# Autodesk Inventor assembly: Foot
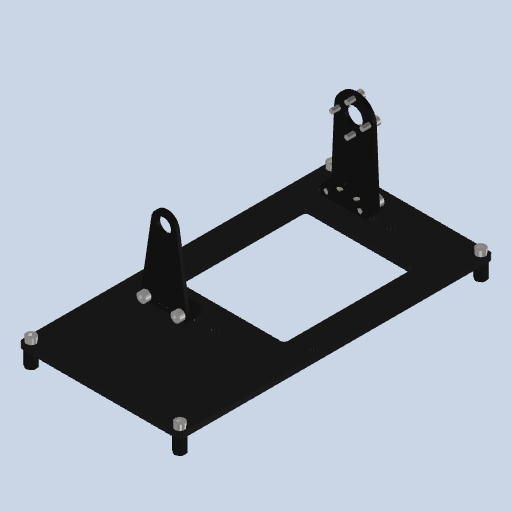
[picture p0: Inventor's stored thumbnail of the model, 512x512]
Saved by Autodesk Inventor 2022 (Build 260153000, 153)
## iProperties
Created: 2022-06-04
Part Number: Foot
Document SubType Name: Assembly
Designer: Masato Kubotera
Author: Masato Kubotera
## Documents named in this file (9)
- C:\Users\MasatoKubotera\Desktop\SUSTAINA-OP\LowerBody\Foot\Foot.iam
- C:\Users\MasatoKubotera\Desktop\SUSTAINA-OP\LowerBody\Foot\Foot_back_frame.ipt
- C:\Users\MasatoKubotera\Desktop\SUSTAINA-OP\LowerBody\Foot\Foot_front_frame.ipt
- C:\Users\MasatoKubotera\Desktop\SUSTAINA-OP\LowerBody\Foot\Foot_root_block.ipt
- C:\Users\MasatoKubotera\Desktop\SUSTAINA-OP\LowerBody\Foot\Sole_frame.ipt
- C:\Users\MasatoKubotera\Desktop\SUSTAINA-OP\ReadyMade\Screw\UC-0308.ipt
- C:\Users\MasatoKubotera\Desktop\SUSTAINA-OP\ReadyMade\Screw\UC-2606.ipt
- C:\Users\MasatoKubotera\Desktop\SUSTAINA-OP\ReadyMade\Spacer\ASL-309BE.ipt
- C:\Users\MasatoKubotera\Desktop\SUSTAINA-OP\ReadyMade\Screw\UC-0310.ipt
## Components (25 placed, 8 different names)
1. Sole_frame:1 — 挿入:1, 挿入:2, 挿入:3, 挿入:4, 挿入:13, 挿入:14, 挿入:15, 挿入:16, 挿入:21, 挿入:22, 挿入:23, 挿入:24, 挿入:25, 挿入:26, 挿入:27, 挿入:28
2. Foot_front_frame:1 — 挿入:5, 挿入:6, メイト:1, メイト:2, 挿入:31, 挿入:32
3. Foot_back_frame:1 — 挿入:7, 挿入:8, 挿入:17, 挿入:18, 挿入:19, 挿入:20, 挿入:29, 挿入:30
4. Foot_root_block:1 — 挿入:1, 挿入:2, 挿入:5, 挿入:6
5. Foot_root_block:2 — 挿入:3, 挿入:4, 挿入:7, 挿入:8
6. ASL-309BE:1 — 挿入:21, メイト:3, 角度:1
7. ASL-309BE:2 — 挿入:22, 角度:2
8. ASL-309BE:3 — 挿入:23, 角度:3
9. ASL-309BE:4 — 挿入:24, 角度:4
10. UC-0308:5 — 挿入:32
11. UC-0308:6 — 挿入:31
12. UC-0308:7 — 挿入:29
13. UC-0308:8 — 挿入:30
14. UC-0310:1 — 挿入:25
15. UC-0310:2 — 挿入:26
16. UC-0310:3 — 挿入:27
17. UC-0310:4 — 挿入:28
18. UC-0308:1 — 挿入:13
19. UC-0308:2 — 挿入:14
20. UC-0308:3 — 挿入:15
21. UC-0308:4 — 挿入:16
22. UC-2606:1 — 挿入:17
23. UC-2606:2 — 挿入:18
24. UC-2606:3 — 挿入:19
25. UC-2606:4 — 挿入:20
## Relationships (35: Insert 28, Angle 4, Mate 3)
- メイト:1 [Mate]: Foot_front_frame:1
- メイト:2 [Mate]: Foot_front_frame:1
- メイト:3 [Mate]: ASL-309BE:1
- 挿入:1 [Insert]: Sole_frame:1 ↔ Foot_root_block:1
- 挿入:2 [Insert]: Sole_frame:1 ↔ Foot_root_block:1
- 挿入:3 [Insert]: Sole_frame:1 ↔ Foot_root_block:2
- 挿入:4 [Insert]: Sole_frame:1 ↔ Foot_root_block:2
- 挿入:5 [Insert]: Foot_front_frame:1 ↔ Foot_root_block:1
- 挿入:6 [Insert]: Foot_front_frame:1 ↔ Foot_root_block:1
- 挿入:7 [Insert]: Foot_back_frame:1 ↔ Foot_root_block:2
- 挿入:8 [Insert]: Foot_back_frame:1 ↔ Foot_root_block:2
- 挿入:13 [Insert]: Sole_frame:1 ↔ UC-0308:1
- 挿入:14 [Insert]: Sole_frame:1 ↔ UC-0308:2
- 挿入:15 [Insert]: Sole_frame:1 ↔ UC-0308:3
- 挿入:16 [Insert]: Sole_frame:1 ↔ UC-0308:4
- 挿入:17 [Insert]: Foot_back_frame:1 ↔ UC-2606:1
- 挿入:18 [Insert]: Foot_back_frame:1 ↔ UC-2606:2
- 挿入:19 [Insert]: Foot_back_frame:1 ↔ UC-2606:3
- 挿入:20 [Insert]: Foot_back_frame:1 ↔ UC-2606:4
- 挿入:21 [Insert]: Sole_frame:1 ↔ ASL-309BE:1
- 挿入:22 [Insert]: Sole_frame:1 ↔ ASL-309BE:2
- 挿入:23 [Insert]: Sole_frame:1 ↔ ASL-309BE:3
- 挿入:24 [Insert]: Sole_frame:1 ↔ ASL-309BE:4
- 挿入:25 [Insert]: Sole_frame:1 ↔ UC-0310:1
- 挿入:26 [Insert]: Sole_frame:1 ↔ UC-0310:2
- 挿入:27 [Insert]: Sole_frame:1 ↔ UC-0310:3
- 挿入:28 [Insert]: Sole_frame:1 ↔ UC-0310:4
- 挿入:29 [Insert]: Foot_back_frame:1 ↔ UC-0308:7
- 挿入:30 [Insert]: Foot_back_frame:1 ↔ UC-0308:8
- 挿入:31 [Insert]: Foot_front_frame:1 ↔ UC-0308:6
- 挿入:32 [Insert]: Foot_front_frame:1 ↔ UC-0308:5
- 角度:1 [Angle] (0 deg): ASL-309BE:1
- 角度:2 [Angle] (0 deg): ASL-309BE:2
- 角度:3 [Angle] (0 deg): ASL-309BE:3
- 角度:4 [Angle] (0 deg): ASL-309BE:4
